# Autodesk Inventor assembly: XCart
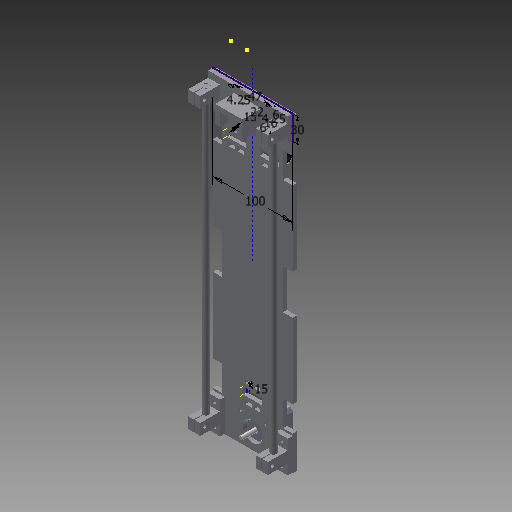
[picture p0: Inventor's stored thumbnail of the model, 512x512]
Saved by Autodesk Inventor 2019 (Build 230136000, 136)
## iProperties
Created: 2019-08-19
Part Number: XCart
Document SubType Name: Assembly
Designer: Bruno
Author: Bruno
## Documents named in this file (8)
- C:\Users\Bruno\Stuff\Ajedrez2\XCart.iam
- C:\Users\Bruno\Stuff\Ajedrez2\XCartFloor.ipt
- C:\Users\Bruno\Stuff\Ajedrez2\Lm8uu.ipt
- C:\Users\Bruno\Stuff\Ajedrez2\17HS10-0704S.ipt
- C:\Users\Bruno\Stuff\Ajedrez2\YPulleySupport.iam
- C:\Users\Bruno\Stuff\Ajedrez2\YRodClamp.ipt
- C:\Users\Bruno\Stuff\Ajedrez2\XCartBeltClamp.ipt
- C:\Users\Bruno\Stuff\Ajedrez2\YRod.ipt
## Components (11 placed, 7 different names)
1. XCartFloor:1 — Mate:1, Mate:2, Mate:4, Mate:5, Mate:6, Rigid:1, Rigid:2, Flush:1, Flush:2, Rigid:3, Rotational:1
2. Lm8uu:1 — Mate:1, Mate:2, Mate:3
3. Lm8uu:2 — Mate:3, Mate:4
4. Lm8uu:3 — Mate:5, Mate:6
5. 17HS10-0704S:1 — Rigid:1
6. YPulleySupport:1 [sub-assembly] — Rigid:2, Rigid:4, Rigid:5
7. YRodClamp:1 — Flush:1, Rigid:3
8. YRodClamp:2 — Rotational:1
9. XCartBeltClamp:1 — Flush:2
10. YRod:1 — Rigid:4
11. YRod:2 — Rigid:5
## Relationships (14: Mate 6, WeldJoint 5, Flush 2, RevoluteJoint 1)
- Mate:1: XCartFloor:1 ↔ Lm8uu:1
- Mate:2: XCartFloor:1 ↔ Lm8uu:1
- Mate:3: Lm8uu:1 ↔ Lm8uu:2
- Mate:4: XCartFloor:1 ↔ Lm8uu:2
- Mate:5: XCartFloor:1 ↔ Lm8uu:3
- Mate:6: XCartFloor:1 ↔ Lm8uu:3
- Rigid:1 [WeldJoint]: XCartFloor:1 ↔ 17HS10-0704S:1
- Rigid:2 [WeldJoint]: XCartFloor:1 ↔ YPulleySupport:1
- Flush:1: XCartFloor:1 ↔ YRodClamp:1
- Flush:2: XCartFloor:1 ↔ XCartBeltClamp:1
- Rigid:3 [WeldJoint]: XCartFloor:1 ↔ YRodClamp:1
- Rotational:1 [RevoluteJoint]: XCartFloor:1 ↔ YRodClamp:2
- Rigid:4 [WeldJoint]: YPulleySupport:1 ↔ YRod:1
- Rigid:5 [WeldJoint]: YPulleySupport:1 ↔ YRod:2
